# Autodesk Inventor assembly: Odometry module
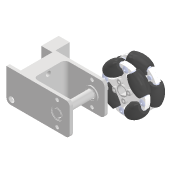
[picture p0: Inventor's stored thumbnail of the model, 180x180]
Saved by Autodesk Inventor 2020 (Build 240168000, 168)
## iProperties
Created: 2019-11-05
Part Number: Odometry module
Document SubType Name: Assembly
Designer: ball
Author: ball
## Documents named in this file (5)
- C:\FTC\FTC8863CAD\2019 Robot\Odoemetry module\Odometry module.iam
- C:\FTC\FTC8863CAD\2019 Robot\Odoemetry module\Odometry_Holder.ipt
- C:\FTC\FTC8863CAD\Actobotics\535 parts\535042.ipt
- C:\FTC\FTC8863CAD\Actobotics\634 parts\634064.ipt
- C:\FTC\FTC8863CAD\2019 Robot\Odoemetry module\wheel_dual.iam
## Components (5 placed, 4 different names)
1. Odometry_Holder:1 — Mate:1, Mate:2, Mate:3, Mate:4, Flush:1
2. 535042:1 — Mate:1, Mate:2
3. 535042:2 — Mate:3, Mate:4, Mate:5
4. 634064:1 — Mate:5, Flush:1, Mate:6
5. wheel_dual:1 [sub-assembly] — Mate:6
## Relationships (7: Mate 6, Flush 1)
- Mate:1: Odometry_Holder:1 ↔ 535042:1
- Mate:2: Odometry_Holder:1 ↔ 535042:1
- Mate:3: Odometry_Holder:1 ↔ 535042:2
- Mate:4: Odometry_Holder:1 ↔ 535042:2
- Mate:5: 535042:2 ↔ 634064:1
- Flush:1: Odometry_Holder:1 ↔ 634064:1
- Mate:6: 634064:1 ↔ wheel_dual:1
